# Autodesk Inventor assembly: Assembly1
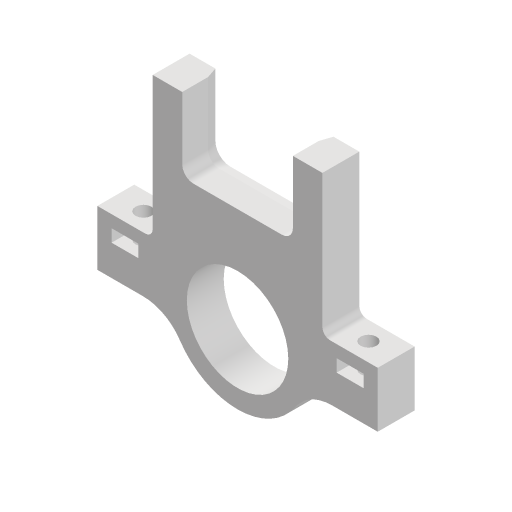
[picture p0: Inventor's stored thumbnail of the model, 512x512]
Saved by Autodesk Inventor 2023.3 (Build 273359000, 359)
## iProperties
Created: 2025-06-02
Part Number: Assembly1
Document SubType Name: Assembly
Designer: David Zindović
Author: David Zindović
## Documents named in this file (3)
- C:\Users\David Zindović\Desktop\Projekti\Bicikl\LIDL U lock\v1.1\Assembly1.iam
- C:\Users\David Zindović\Desktop\Projekti\Bicikl\LIDL U lock\v1.1\Part1.ipt
- C:\Users\David Zindović\Desktop\Projekti\Bicikl\LIDL U lock\v1.1\Part2.ipt
## Components (2 placed, 2 different names)
1. Part1:1 — Mate:1, Mate:2, Mate:3
2. Part2:1 — Mate:1, Mate:2, Mate:3
## Relationships (3: Mate 3)
- Mate:1: Part1:1 ↔ Part2:1
- Mate:2: Part1:1 ↔ Part2:1
- Mate:3: Part1:1 ↔ Part2:1
